# Autodesk Inventor assembly: Feeder Assembly V2
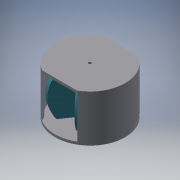
[picture p0: Inventor's stored thumbnail of the model, 180x180]
Saved by Autodesk Inventor 2017 (Build 210142000, 142)
## iProperties
Created: 2019-01-21
Part Number: Feeder Assembly V2
Document SubType Name: Assembly
Designer: Matt
Author: Matt
## Documents named in this file (4)
- C:\Users\Matt\Documents\Cat Feeder\Feeder Assembly V2.iam
- C:\Users\Matt\Documents\Cat Feeder\Gear Container V2.ipt
- C:\Users\Matt\Documents\Cat Feeder\Dispensing Gear V2.ipt
- C:\Users\Matt\Documents\Cat Feeder\Gear Container Lid V2.ipt
## Components (3 placed, 3 different names)
1. Gear Container V2:1 — Mate:1, Mate:2, Mate:3, Mate:4
2. Dispensing Gear V2:1 — Mate:1
3. Gear Container Lid V2:1 — Mate:2, Mate:3, Mate:4
## Relationships (4: Mate 4)
- Mate:1: Gear Container V2:1 ↔ Dispensing Gear V2:1
- Mate:2: Gear Container V2:1 ↔ Gear Container Lid V2:1
- Mate:3: Gear Container V2:1 ↔ Gear Container Lid V2:1
- Mate:4: Gear Container V2:1 ↔ Gear Container Lid V2:1
